# Autodesk Inventor assembly: MovingPlate
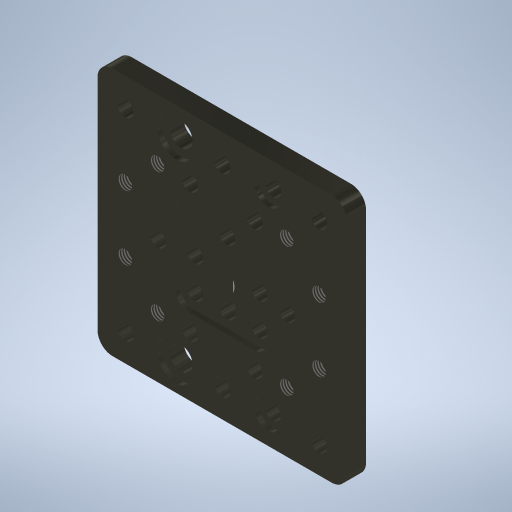
[picture p0: Inventor's stored thumbnail of the model, 512x512]
Saved by Autodesk Inventor 2024.2 (Build 282272000, 272)
## iProperties
Created: 2024-08-27
Part Number: MovingPlate
Document SubType Name: Assembly
Designer: Admin
Author: Admin
## Documents named in this file (4)
- C:\Users\Admin\Documents\GitHub\RobotCartesiano\DiseñoBrazo\AluminumProfiles\AxisZ\LinearActuator\MovingPlate\MovingPlate.iam
- C:\Users\Admin\Documents\GitHub\RobotCartesiano\DiseñoBrazo\AluminumProfiles\AxisZ\LinearActuator\MovingPlate\AntiBacklashBlock.ipt
- C:\Users\Admin\Documents\GitHub\RobotCartesiano\DiseñoBrazo\AluminumProfiles\AxisZ\LinearActuator\MovingPlate\AluminiumSpacer3mm.ipt
- C:\Users\Admin\Documents\GitHub\RobotCartesiano\DiseñoBrazo\AluminumProfiles\AxisZ\LinearActuator\MovingPlate\C-BeamPlate.ipt
## Components (4 placed, 3 different names)
1. AntiBacklashBlock:1 — Mate:1, Mate:2, Mate:3, Mate:4
2. AluminiumSpacer3mm:1 — Mate:3, Mate:4, Mate:5, Mate:7
3. AluminiumSpacer3mm:2 — Mate:1, Mate:2, Mate:6
4. C-BeamPlate:1 — Mate:5, Mate:6, Mate:7
## Relationships (7: Mate 7)
- Mate:1: AntiBacklashBlock:1 ↔ AluminiumSpacer3mm:2
- Mate:2: AntiBacklashBlock:1 ↔ AluminiumSpacer3mm:2
- Mate:3: AntiBacklashBlock:1 ↔ AluminiumSpacer3mm:1
- Mate:4: AntiBacklashBlock:1 ↔ AluminiumSpacer3mm:1
- Mate:5: AluminiumSpacer3mm:1 ↔ C-BeamPlate:1
- Mate:6: AluminiumSpacer3mm:2 ↔ C-BeamPlate:1
- Mate:7: AluminiumSpacer3mm:1 ↔ C-BeamPlate:1
